# Autodesk Inventor assembly: y-platform
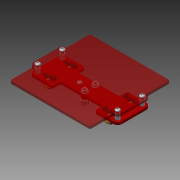
[picture p0: Inventor's stored thumbnail of the model, 180x180]
Saved by Autodesk Inventor 2013 (Build 170138000, 138)
## iProperties
Created: 2015-02-19
Part Number: y-platform
Document SubType Name: Assembly
Designer: Noa Izumi
Author: Noa Izumi
## Documents named in this file (13)
- C:\reprap\TinyBoy_v3_20150221\assembly y.iam
- C:\reprap\TinyBoy_v3_20150221\plastic_part_12.ipt
- C:\reprap\TinyBoy_v3_20150221\plastic_part_13.ipt
- C:\reprap\TinyBoy_v3_20150221\screw_M3_16_hex.ipt
- C:\reprap\TinyBoy_v3_20150221\screw_M3_12_hex.ipt
- C:\reprap\TinyBoy_v3_20150221\washer_M3.ipt
- C:\reprap\TinyBoy_v3_20150221\screw_M3_6_hex.ipt
- C:\reprap\TinyBoy_v3_20150221\nut_rod_M3_6.ipt
- C:\reprap\TinyBoy_v3_20150221\nut_M3.ipt
- C:\reprap\TinyBoy_v3_20150221\ring_488.ipt
- C:\reprap\TinyBoy_v3_20150221\plastic_part_11.ipt
- C:\reprap\TinyBoy_v3_20150221\fastener_01.ipt
- C:\reprap\TinyBoy_v3_20150221\bearing_603zz.ipt
## Components (34 placed, 12 different names)
1. plastic_part_12:1 — 插入:1, 插入:2, 插入:5, 插入:6, 插入:7, 插入:8, 插入:9, 插入:18, 插入:20, 貼合:1, 貼合:2, 貼合:3, 貼合:4, 相切:1, 相切:2, 相切:3, 相切:4, 相切:5, 相切:6, 相切:7, 相切:8, 角度:5, 角度:6, 角度:7, 角度:8, 插入:32, 插入:33, 插入:34, 插入:35, 角度:9, 角度:10, 角度:11, 角度:12
2. plastic_part_13:1 — 插入:1, 插入:2, 插入:14, 插入:15
3. screw_M3_16_hex:1 — 插入:3
4. screw_M3_16_hex:2 — 插入:4
5. screw_M3_12_hex:1 — 插入:5
6. washer_M3:1 — 插入:15, 插入:17
7. washer_M3:2 — 插入:14, 插入:16
8. bearing_603zz:1 — 插入:3, 插入:16
9. bearing_603zz:2 — 插入:4, 插入:17
10. screw_M3_6_hex:1 — 插入:24
11. screw_M3_6_hex:2 — 插入:9
12. screw_M3_6_hex:3 — 插入:7
13. screw_M3_6_hex:4 — 插入:8
14. screw_M3_6_hex:5 — 插入:27
15. screw_M3_6_hex:6 — 插入:26
16. screw_M3_6_hex:7 — 插入:25
17. screw_M3_6_hex:8 — 插入:6
18. nut_rod_M3_6:1 — 插入:33, 插入:36, 角度:11
19. nut_rod_M3_6:2 — 插入:32, 插入:37, 角度:12
20. nut_rod_M3_6:3 — 插入:34, 角度:10
21. nut_rod_M3_6:4 — 插入:35, 角度:9
22. washer_M3:3 — 插入:20, 插入:21
23. washer_M3:4 — 插入:18, 插入:19
24. nut_M3:1 — 插入:21
25. nut_M3:2 — 插入:19
26. ring_488:1 — 貼合:1, 相切:4, 相切:8, 插入:29
27. ring_488:2 — 貼合:2, 相切:3, 相切:7, 插入:28
28. ring_488:3 — 貼合:3, 相切:2, 相切:6, 插入:30
29. ring_488:4 — 貼合:4, 相切:1, 相切:5, 插入:31
30. plastic_part_11:1 — 插入:24, 插入:25, 插入:26, 插入:27, 插入:36, 插入:37
31. fastener_01:1 — 插入:28, 角度:8
32. fastener_01:2 — 插入:29, 角度:7
33. fastener_01:3 — 插入:31, 角度:5
34. fastener_01:4 — 插入:30, 角度:6
## Relationships (51: Insert 31, Tangent 8, Angle 8, Mate 4)
- 插入:1 [Insert]: plastic_part_12:1 ↔ plastic_part_13:1
- 插入:2 [Insert]: plastic_part_12:1 ↔ plastic_part_13:1
- 插入:3 [Insert]: screw_M3_16_hex:1 ↔ bearing_603zz:1
- 插入:4 [Insert]: screw_M3_16_hex:2 ↔ bearing_603zz:2
- 插入:5 [Insert]: plastic_part_12:1 ↔ screw_M3_12_hex:1
- 插入:6 [Insert]: plastic_part_12:1 ↔ screw_M3_6_hex:8
- 插入:7 [Insert]: plastic_part_12:1 ↔ screw_M3_6_hex:3
- 插入:8 [Insert]: plastic_part_12:1 ↔ screw_M3_6_hex:4
- 插入:9 [Insert]: plastic_part_12:1 ↔ screw_M3_6_hex:2
- 插入:14 [Insert]: plastic_part_13:1 ↔ washer_M3:2
- 插入:15 [Insert]: plastic_part_13:1 ↔ washer_M3:1
- 插入:16 [Insert]: washer_M3:2 ↔ bearing_603zz:1
- 插入:17 [Insert]: washer_M3:1 ↔ bearing_603zz:2
- 插入:18 [Insert]: plastic_part_12:1 ↔ washer_M3:4
- 插入:19 [Insert]: washer_M3:4 ↔ nut_M3:2
- 插入:20 [Insert]: plastic_part_12:1 ↔ washer_M3:3
- 插入:21 [Insert]: washer_M3:3 ↔ nut_M3:1
- 貼合:1 [Mate]: plastic_part_12:1 ↔ ring_488:1
- 貼合:2 [Mate]: plastic_part_12:1 ↔ ring_488:2
- 貼合:3 [Mate]: plastic_part_12:1 ↔ ring_488:3
- 貼合:4 [Mate]: plastic_part_12:1 ↔ ring_488:4
- 相切:1 [Tangent]: plastic_part_12:1 ↔ ring_488:4
- 相切:2 [Tangent]: plastic_part_12:1 ↔ ring_488:3
- 相切:3 [Tangent]: plastic_part_12:1 ↔ ring_488:2
- 相切:4 [Tangent]: plastic_part_12:1 ↔ ring_488:1
- 相切:5 [Tangent]: plastic_part_12:1 ↔ ring_488:4
- 相切:6 [Tangent]: plastic_part_12:1 ↔ ring_488:3
- 相切:7 [Tangent]: plastic_part_12:1 ↔ ring_488:2
- 相切:8 [Tangent]: plastic_part_12:1 ↔ ring_488:1
- 插入:24 [Insert]: screw_M3_6_hex:1 ↔ plastic_part_11:1
- 插入:25 [Insert]: screw_M3_6_hex:7 ↔ plastic_part_11:1
- 插入:26 [Insert]: screw_M3_6_hex:6 ↔ plastic_part_11:1
- 插入:27 [Insert]: screw_M3_6_hex:5 ↔ plastic_part_11:1
- 插入:28 [Insert] (2.75 mm): ring_488:2 ↔ fastener_01:1
- 插入:29 [Insert] (2.75 mm): ring_488:1 ↔ fastener_01:2
- 插入:30 [Insert] (2.75 mm): ring_488:3 ↔ fastener_01:4
- 插入:31 [Insert] (2.75 mm): ring_488:4 ↔ fastener_01:3
- 角度:5 [Angle] (0 deg): plastic_part_12:1 ↔ fastener_01:3
- 角度:6 [Angle] (0 deg): plastic_part_12:1 ↔ fastener_01:4
- 角度:7 [Angle] (0 deg): plastic_part_12:1 ↔ fastener_01:2
- 角度:8 [Angle] (0 deg): plastic_part_12:1 ↔ fastener_01:1
- 插入:32 [Insert]: plastic_part_12:1 ↔ nut_rod_M3_6:2
- 插入:33 [Insert]: plastic_part_12:1 ↔ nut_rod_M3_6:1
- 插入:34 [Insert]: plastic_part_12:1 ↔ nut_rod_M3_6:3
- 插入:35 [Insert]: plastic_part_12:1 ↔ nut_rod_M3_6:4
- 插入:36 [Insert]: nut_rod_M3_6:1 ↔ plastic_part_11:1
- 插入:37 [Insert]: nut_rod_M3_6:2 ↔ plastic_part_11:1
- 角度:9 [Angle] (0 deg): plastic_part_12:1 ↔ nut_rod_M3_6:4
- 角度:10 [Angle] (0 deg): plastic_part_12:1 ↔ nut_rod_M3_6:3
- 角度:11 [Angle] (0 deg): plastic_part_12:1 ↔ nut_rod_M3_6:1
- 角度:12 [Angle] (0 deg): plastic_part_12:1 ↔ nut_rod_M3_6:2
